# Autodesk Inventor assembly: bevel gear with clamping hub
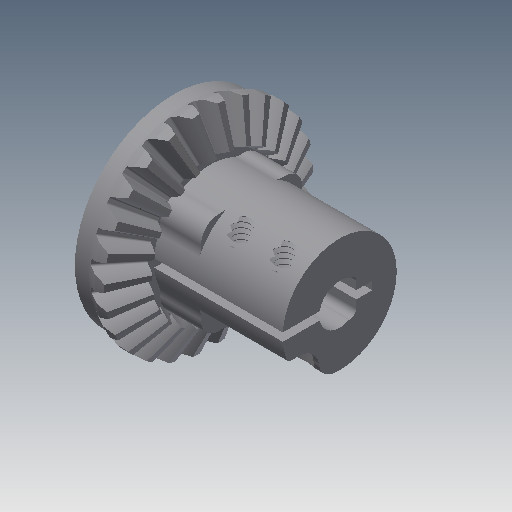
[picture p0: Inventor's stored thumbnail of the model, 512x512]
Saved by Autodesk Inventor 2019 (Build 230136000, 136)
## iProperties
Created: 2019-09-29
Part Number: bevel gear with clamping hub
Document SubType Name: Assembly
Designer: ball
Author: ball
## Documents named in this file (4)
- C:\FTC\FTC8863CAD\2019 Robot\Mecanum Drive Train\bevel gear with clamping hub.iam
- C:\FTC\FTC8863CAD\Actobotics\615 parts\615460.ipt
- C:\FTC\FTC8863CAD\Actobotics\545 parts\545309.ipt
- C:\FTC\FTC8863CAD\Actobotics\632 parts\632108.ipt
## Components (6 placed, 3 different names)
1. 615460:1 — Mate:1, Mate:2, Mate:3, Mate:4, Mate:5, Mate:6, Mate:7, Mate:8
2. 545309:1 — Mate:1, Mate:2, Mate:3, Mate:9, Mate:10, Mate:11
3. 632108:1 — Mate:4, Mate:5
4. 632108:2 — Mate:7, Mate:11
5. 632108:3 — Mate:8, Mate:10
6. 632108:4 — Mate:6, Mate:9
## Relationships (11: Mate 11)
- Mate:1: 615460:1 ↔ 545309:1
- Mate:2: 615460:1 ↔ 545309:1
- Mate:3: 615460:1 ↔ 545309:1
- Mate:4: 615460:1 ↔ 632108:1
- Mate:5: 615460:1 ↔ 632108:1
- Mate:6: 615460:1 ↔ 632108:4
- Mate:7: 615460:1 ↔ 632108:2
- Mate:8: 615460:1 ↔ 632108:3
- Mate:9: 545309:1 ↔ 632108:4
- Mate:10: 545309:1 ↔ 632108:3
- Mate:11: 545309:1 ↔ 632108:2
